# Autodesk Inventor assembly: Body
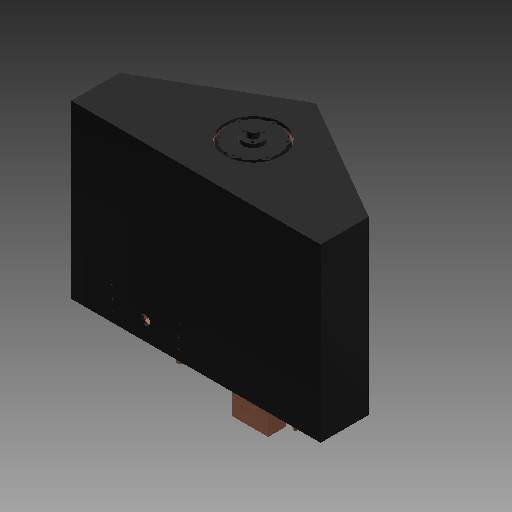
[picture p0: Inventor's stored thumbnail of the model, 512x512]
Saved by Autodesk Inventor 2017 (Build 210142000, 142)
## iProperties
Created: 2018-10-18
Part Number: Body
Document SubType Name: Assembly
Designer: Dell
Author: Dell
## Documents named in this file (6)
- C:\Users\Dell\Documents\GitHub\tr2\Body\Body.iam
- C:\Users\Dell\Documents\GitHub\tr2\Body\Body Cover Assembly.iam
- C:\Users\Dell\Documents\GitHub\tr2\Body\Body Chassis Assembly.iam
- C:\Users\Dell\Documents\GitHub\tr2\Arm Actuator\Arm Actuator.iam
- C:\Users\Dell\Documents\GitHub\tr2\Body\BO13.ipt
- C:\Users\Dell\Documents\GitHub\tr2\Body\CA01.ipt
## Components (5 placed, 5 different names)
1. Body Cover Assembly:1 [sub-assembly] — Mate:72, Flush:1, Mate:78
2. Body Chassis Assembly:1 [sub-assembly] — Mate:72, Mate:78, Mate:79, Mate:81, Mate:82, Mate:83, Mate:84, Mate:85, Mate:86, Mate:87, Flush:2
3. Arm Actuator:1 [sub-assembly] — Mate:69, Mate:70, Flush:1, Mate:74, Mate:75, Mate:76, Mate:77
4. BO13:1 — Mate:69, Mate:70, Mate:74, Mate:75, Mate:76, Mate:77, Mate:79, Mate:81
5. CA01:1 — Mate:82, Mate:83, Mate:84
## Relationships (18: Mate 16, Flush 2)
- Mate:69: Arm Actuator:1 ↔ BO13:1
- Mate:70: Arm Actuator:1 ↔ BO13:1
- Mate:72: Body Cover Assembly:1 ↔ Body Chassis Assembly:1
- Flush:1: Body Cover Assembly:1 ↔ Arm Actuator:1
- Mate:74: Arm Actuator:1 ↔ BO13:1
- Mate:75: Arm Actuator:1 ↔ BO13:1
- Mate:76: Arm Actuator:1 ↔ BO13:1
- Mate:77: Arm Actuator:1 ↔ BO13:1
- Mate:78: Body Cover Assembly:1 ↔ Body Chassis Assembly:1
- Mate:79: Body Chassis Assembly:1 ↔ BO13:1
- Mate:81: Body Chassis Assembly:1 ↔ BO13:1
- Mate:82: Body Chassis Assembly:1 ↔ CA01:1
- Mate:83: Body Chassis Assembly:1 ↔ CA01:1
- Mate:84: Body Chassis Assembly:1 ↔ CA01:1
- Mate:85: Body Chassis Assembly:1
- Mate:86: Body Chassis Assembly:1
- Mate:87: Body Chassis Assembly:1
- Flush:2: Body Chassis Assembly:1
